# Autodesk Inventor assembly: CHANNEL_LEG ASSEMBLY
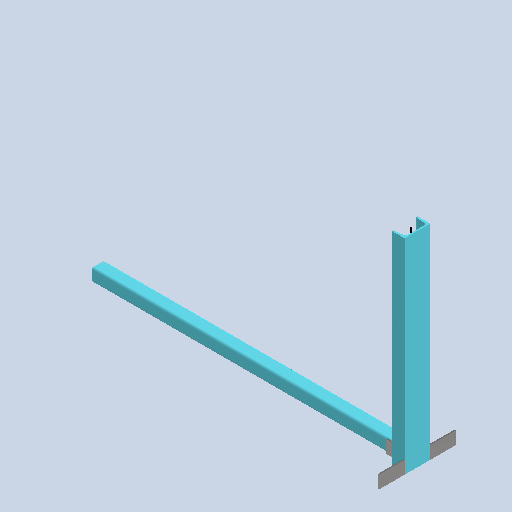
[picture p0: Inventor's stored thumbnail of the model, 512x512]
Saved by Autodesk Inventor 2023 (Build 270158000, 158)
## iProperties
Created: 2025-04-10
Part Number: CHANNEL_LEG ASSEMBLY
Document SubType Name: Assembly
Designer: NELLY NDUNG'U
Author: NELLY NDUNG'U
## Documents named in this file (6)
- N:\NAKUJA\CAD FILES\AIRFRAME\LP003\CHANNEL_LEG ASSEMBLY.iam
- N:\NAKUJA\CAD FILES\AIRFRAME\LP003\U_SECTION_50.iam
- N:\NAKUJA\CAD FILES\AIRFRAME\LP003\LEG_50.iam
- N:\NAKUJA\CAD FILES\AIRFRAME\LP003\LEG_ATTACHMENT1.ipt
- C:\Users\User\Documents\Inventor\Content Center Files\R2023\en-US\ANSI B18.2.3.5M\ANSI B18.2.3.5M - M16 x 2 x 80.ipt
- C:\Users\User\Documents\Inventor\Content Center Files\R2023\en-US\ANSI B 18.2.4.1 M(1)\ANSI B 18.2.4.1 M - M16 x 2Style 1.ipt
## Components (7 placed, 5 different names)
1. U_SECTION_50:1 [sub-assembly] — Mate:1, Flush:1, Flush:2, Mate:2, Flush:3, Flush:4, Mate:3, Mate:4, Flush:5, Mate:5, Insert:1
2. LEG_ATTACHMENT1:1 — Mate:1, Flush:1, Flush:3
3. LEG_ATTACHMENT1:2 — Flush:2, Mate:2, Flush:4
4. LEG_ATTACHMENT1:3 — Mate:3, Mate:4, Flush:5, Mate:6, Flush:6, Insert:2
5. LEG_50:1 [sub-assembly] — Mate:5, Mate:6, Flush:6
6. Hex Bolt - Metric M16 x 2 x 80:1 — Insert:1
7. Hex Nut Metric M16 x 2:1 — Insert:2
## Relationships (14: Mate 6, Flush 6, Insert 2)
- Mate:1: U_SECTION_50:1 ↔ LEG_ATTACHMENT1:1
- Flush:1: U_SECTION_50:1 ↔ LEG_ATTACHMENT1:1
- Flush:2: U_SECTION_50:1 ↔ LEG_ATTACHMENT1:2
- Mate:2: U_SECTION_50:1 ↔ LEG_ATTACHMENT1:2
- Flush:3: U_SECTION_50:1 ↔ LEG_ATTACHMENT1:1
- Flush:4: U_SECTION_50:1 ↔ LEG_ATTACHMENT1:2
- Mate:3: U_SECTION_50:1 ↔ LEG_ATTACHMENT1:3
- Mate:4 (-65 mm): U_SECTION_50:1 ↔ LEG_ATTACHMENT1:3
- Flush:5: U_SECTION_50:1 ↔ LEG_ATTACHMENT1:3
- Mate:5 (5 mm): U_SECTION_50:1 ↔ LEG_50:1
- Mate:6: LEG_ATTACHMENT1:3 ↔ LEG_50:1
- Flush:6: LEG_ATTACHMENT1:3 ↔ LEG_50:1
- Insert:1: U_SECTION_50:1 ↔ Hex Bolt - Metric M16 x 2 x 80:1
- Insert:2: LEG_ATTACHMENT1:3 ↔ Hex Nut Metric M16 x 2:1
